# Autodesk Inventor assembly: sestava tělo estonsko s plechem otočené motory
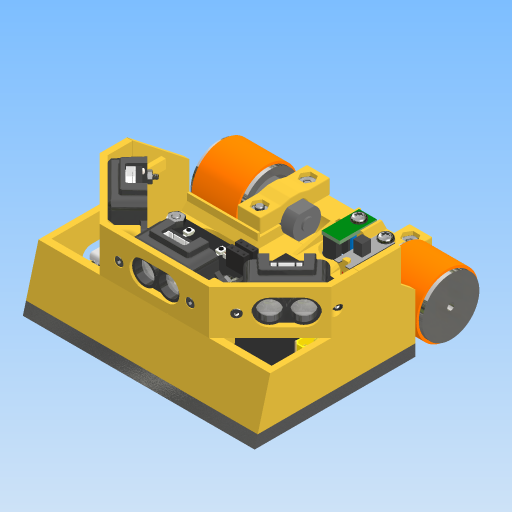
[picture p0: Inventor's stored thumbnail of the model, 512x512]
Saved by Autodesk Inventor 2024.2 (Build 282272000, 272)
## iProperties
Created: 2023-11-14
Part Number: sestava tělo estonsko s plechem otočené motory
Document SubType Name: Assembly
Designer: Simak
Author: Simak
## Documents named in this file (21)
- C:\Users\MenMe\Рабочий стол\GitHub\RoboCop\- 3D -\wip\Tělo s plechem\sestava tělo estonsko s plechem otočené motory.iam
- C:\Users\MenMe\Рабочий стол\GitHub\RoboCop\- 3D -\wip\Tělo s plechem\tělo estonsko s plechem otočené motory.ipt
- C:\Users\MenMe\Рабочий стол\GitHub\RoboCop\- 3D -\mech._parts\plech.ipt
- C:\Users\MenMe\Рабочий стол\GitHub\RoboCop\- 3D -\el._parts\sumec_smd.iam
- C:\Users\MenMe\Рабочий стол\GitHub\RoboCop\- 3D -\wip\Sestava TF-Luna a držáku.iam
- C:\Users\MenMe\Рабочий стол\GitHub\RoboCop\- 3D -\el._parts\qre_module.ipt
- C:\Users\MenMe\Рабочий стол\GitHub\RoboCop\- 3D -\el._parts\switch.ipt
- C:\Users\MenMe\Рабочий стол\GitHub\RoboCop\- 3D -\el._parts\GA12-N20_Motor.ipt
- C:\Users\MenMe\Рабочий стол\GitHub\RoboCop\- 3D -\mech._parts\wheel+silicon.ipt
- C:\Users\MenMe\Рабочий стол\GitHub\RoboCop\- 3D -\mech._parts\motor_C_clamp_nutt_motor_otoceny.ipt
- C:\Users\MenMe\Рабочий стол\GitHub\RoboCop\- 3D -\screws+nuts\Šrouby\M3_kuzel_torx\torx_socket_countersunk_flat_head_M3x18.ipt
- C:\Users\MenMe\Рабочий стол\GitHub\RoboCop\- 3D -\screws+nuts\matky\M3 Nut.ipt
- C:\Users\MenMe\Рабочий стол\GitHub\RoboCop\- 3D -\screws+nuts\Šrouby\M3_kuzel_torx\torx_socket_countersunk_flat_head_M3x08.ipt
- C:\Users\MenMe\Рабочий стол\GitHub\RoboCop\- 3D -\screws+nuts\Šrouby\M3_koule_torx\torx_socket_button_head_M3x08.ipt
- C:\Users\MenMe\Рабочий стол\GitHub\RoboCop\- 3D -\screws+nuts\Šrouby\M3_kuzel_torx\torx_socket_countersunk_flat_head_M3x12.ipt
- C:\Users\MenMe\Рабочий стол\GitHub\RoboCop\- 3D -\screws+nuts\Šrouby\M3_koule_torx\torx_socket_button_head_M3x10.ipt
- C:\Users\MenMe\Рабочий стол\GitHub\RoboCop\- 3D -\screws+nuts\Šrouby\M2_valec_imbus\M2 x 0.4mm Thread 16mm LONG SOCKET HEAD CAP SCREW.ipt
- C:\Users\MenMe\Рабочий стол\GitHub\RoboCop\- 3D -\screws+nuts\Šrouby\M2_valec_imbus\M2 x 0.4mm Thread 12mm LONG SOCKET HEAD CAP SCREW.ipt
- C:\Users\MenMe\Рабочий стол\GitHub\RoboCop\- 3D -\el._parts\connectors\XT30\XT30_Stecker.ipt
- C:\Users\MenMe\Рабочий стол\GitHub\RoboCop\- 3D -\screws+nuts\matky\M2 x 0.4mm Thread HEX NUT.ipt
- C:\Users\MenMe\Рабочий стол\GitHub\RoboCop\- 3D -\mech._parts\oddělovací plocha.ipt
## Components (50 placed, 20 different names)
1. tělo estonsko s plechem otočené motory:1 — Mate:1, Flush:1, Flush:2, Mate:2, Insert:1, Insert:2, Mate:3, Mate:4, Flush:3, Insert:3, Mate:5, Mate:6, Mate:7, Mate:8, Mate:10, Mate:11, Mate:12, Mate:13, Mate:14, Mate:15, Flush:4, Flush:5, Mate:19, Insert:4, Mate:21, Insert:5, Insert:8, Insert:9, Mate:28, Mate:39, Mate:40, Insert:27, Insert:28, Mate:41, Mate:42, Insert:34, Mate:45, Mate:47
2. plech:1 — Mate:1, Flush:1, Flush:2, Insert:6, Insert:7, Insert:11, Insert:12, Insert:13, Insert:14, Mate:46, Insert:35
3. sumec_smd:1 [sub-assembly] — Mate:2, Insert:1, Insert:2, Mate:34, Mate:35, Mate:36, Insert:23, Insert:24, Insert:25, Insert:26
4. Sestava TF-Luna a držáku:1 [sub-assembly] — Mate:3, Mate:4, Flush:3, Mate:30, Mate:31, Mate:32, Mate:33, Insert:15, Insert:16, Insert:17, Insert:18, Insert:19, Insert:20, Mate:44, Insert:29, Insert:30, Insert:31, Insert:32, Insert:33
5. qre_module:1 — Insert:3, Mate:5, Insert:10
6. switch:1 — Mate:6, Mate:7, Mate:8, Mate:29
7. GA12-N20_Motor:1 — Mate:13, Mate:14, Mate:15, Mate:17, Mate:20
8. GA12-N20_Motor:2 — Mate:10, Mate:11, Mate:12, Mate:16, Mate:18
9. wheel+silicon:1 — Flush:5, Mate:17
10. wheel+silicon:2 — Flush:4, Mate:16
11. motor_C_clamp_nutt_motor_otoceny:1 — Mate:18, Mate:19, Insert:4, Mate:22, Mate:24, Insert:21, Mate:37
12. motor_C_clamp_nutt_motor_otoceny:2 — Mate:20, Mate:21, Insert:5, Mate:25, Mate:27, Insert:22, Mate:38
13. torx_socket_countersunk_flat_head_M3x18:1 — Insert:7, Mate:23
14. torx_socket_countersunk_flat_head_M3x18:2 — Insert:6, Mate:26
15. M3 Nut:6 — Mate:25, Mate:26, Mate:27
16. M3 Nut:8 — Mate:22, Mate:23, Mate:24
17. torx_socket_countersunk_flat_head_M3x08:1 — Insert:9
18. torx_socket_countersunk_flat_head_M3x08:2 — Insert:8
19. torx_socket_button_head_M3x08:1 — Insert:10
20. torx_socket_button_head_M3x08:2 — Mate:28, Mate:29
21. torx_socket_countersunk_flat_head_M3x12:1 — Insert:14
22. torx_socket_countersunk_flat_head_M3x12:2 — Insert:12
23. torx_socket_countersunk_flat_head_M3x12:3 — Insert:13
24. torx_socket_countersunk_flat_head_M3x12:4 — Insert:11
25. torx_socket_button_head_M3x10:1 — Mate:31, Mate:32
26. torx_socket_button_head_M3x10:2 — Mate:30, Mate:33
27. M2 x 0.4mm Thread 16mm LONG SOCKET HEAD CAP SCREW:1 — Insert:18
28. M2 x 0.4mm Thread 16mm LONG SOCKET HEAD CAP SCREW:2 — Insert:17
29. M2 x 0.4mm Thread 16mm LONG SOCKET HEAD CAP SCREW:3 — Insert:16
30. M2 x 0.4mm Thread 16mm LONG SOCKET HEAD CAP SCREW:4 — Insert:15
31. M2 x 0.4mm Thread 12mm LONG SOCKET HEAD CAP SCREW:1 — Insert:20
32. M2 x 0.4mm Thread 12mm LONG SOCKET HEAD CAP SCREW:2 — Insert:19, Mate:43
33. XT30_Stecker:1 — Mate:34, Mate:35, Mate:36
34. M3 Nut:9 — Insert:24
35. M3 Nut:10 — Insert:23
36. M3 Nut:11 — Mate:39, Mate:40
37. M3 Nut:12 — Insert:21, Mate:37
38. M3 Nut:13 — Insert:22, Mate:38
39. M3 Nut:14 — Insert:25
40. M3 Nut:15 — Insert:26
41. M3 Nut:16 — Insert:28, Mate:41
42. M3 Nut:17 — Insert:27, Mate:42
43. M2 x 0.4mm Thread HEX NUT:1 — Insert:31
44. M2 x 0.4mm Thread HEX NUT:2 — Insert:30
45. M2 x 0.4mm Thread HEX NUT:3 — Insert:33
46. M2 x 0.4mm Thread HEX NUT:4 — Insert:32
47. M2 x 0.4mm Thread HEX NUT:5 — Insert:29
48. M2 x 0.4mm Thread HEX NUT:6 — Mate:43, Mate:44
49. M3 Nut:18 — Insert:34, Mate:45
50. oddělovací plocha:1 — Mate:46, Insert:35, Mate:47
## Relationships (86: Mate 46, Insert 35, Flush 5)
- Mate:1: tělo estonsko s plechem otočené motory:1 ↔ plech:1
- Flush:1: tělo estonsko s plechem otočené motory:1 ↔ plech:1
- Flush:2: tělo estonsko s plechem otočené motory:1 ↔ plech:1
- Mate:2: tělo estonsko s plechem otočené motory:1 ↔ sumec_smd:1
- Insert:1: tělo estonsko s plechem otočené motory:1 ↔ sumec_smd:1
- Insert:2: tělo estonsko s plechem otočené motory:1 ↔ sumec_smd:1
- Mate:3: tělo estonsko s plechem otočené motory:1 ↔ Sestava TF-Luna a držáku:1
- Mate:4: tělo estonsko s plechem otočené motory:1 ↔ Sestava TF-Luna a držáku:1
- Flush:3: tělo estonsko s plechem otočené motory:1 ↔ Sestava TF-Luna a držáku:1
- Insert:3: tělo estonsko s plechem otočené motory:1 ↔ qre_module:1
- Mate:5: tělo estonsko s plechem otočené motory:1 ↔ qre_module:1
- Mate:6: tělo estonsko s plechem otočené motory:1 ↔ switch:1
- Mate:7: tělo estonsko s plechem otočené motory:1 ↔ switch:1
- Mate:8: tělo estonsko s plechem otočené motory:1 ↔ switch:1
- Mate:10: tělo estonsko s plechem otočené motory:1 ↔ GA12-N20_Motor:2
- Mate:11: tělo estonsko s plechem otočené motory:1 ↔ GA12-N20_Motor:2
- Mate:12: tělo estonsko s plechem otočené motory:1 ↔ GA12-N20_Motor:2
- Mate:13: tělo estonsko s plechem otočené motory:1 ↔ GA12-N20_Motor:1
- Mate:14: tělo estonsko s plechem otočené motory:1 ↔ GA12-N20_Motor:1
- Mate:15: tělo estonsko s plechem otočené motory:1 ↔ GA12-N20_Motor:1
- Flush:4: tělo estonsko s plechem otočené motory:1 ↔ wheel+silicon:2
- Mate:16: GA12-N20_Motor:2 ↔ wheel+silicon:2
- Flush:5: tělo estonsko s plechem otočené motory:1 ↔ wheel+silicon:1
- Mate:17: GA12-N20_Motor:1 ↔ wheel+silicon:1
- Mate:18: GA12-N20_Motor:2 ↔ motor_C_clamp_nutt_motor_otoceny:1
- Mate:19: tělo estonsko s plechem otočené motory:1 ↔ motor_C_clamp_nutt_motor_otoceny:1
- Insert:4: tělo estonsko s plechem otočené motory:1 ↔ motor_C_clamp_nutt_motor_otoceny:1
- Mate:20: GA12-N20_Motor:1 ↔ motor_C_clamp_nutt_motor_otoceny:2
- Mate:21: tělo estonsko s plechem otočené motory:1 ↔ motor_C_clamp_nutt_motor_otoceny:2
- Insert:5: tělo estonsko s plechem otočené motory:1 ↔ motor_C_clamp_nutt_motor_otoceny:2
- Insert:6: plech:1 ↔ torx_socket_countersunk_flat_head_M3x18:2
- Insert:7: plech:1 ↔ torx_socket_countersunk_flat_head_M3x18:1
- Mate:22: motor_C_clamp_nutt_motor_otoceny:1 ↔ M3 Nut:8
- Mate:23: torx_socket_countersunk_flat_head_M3x18:1 ↔ M3 Nut:8
- Mate:24: motor_C_clamp_nutt_motor_otoceny:1 ↔ M3 Nut:8
- Mate:25: motor_C_clamp_nutt_motor_otoceny:2 ↔ M3 Nut:6
- Mate:26: torx_socket_countersunk_flat_head_M3x18:2 ↔ M3 Nut:6
- Mate:27: motor_C_clamp_nutt_motor_otoceny:2 ↔ M3 Nut:6
- Insert:8: tělo estonsko s plechem otočené motory:1 ↔ torx_socket_countersunk_flat_head_M3x08:2
- Insert:9: tělo estonsko s plechem otočené motory:1 ↔ torx_socket_countersunk_flat_head_M3x08:1
- Insert:10: qre_module:1 ↔ torx_socket_button_head_M3x08:1
- Mate:28: tělo estonsko s plechem otočené motory:1 ↔ torx_socket_button_head_M3x08:2
- Mate:29: switch:1 ↔ torx_socket_button_head_M3x08:2
- Insert:11: plech:1 ↔ torx_socket_countersunk_flat_head_M3x12:4
- Insert:12: plech:1 ↔ torx_socket_countersunk_flat_head_M3x12:2
- Insert:13: plech:1 ↔ torx_socket_countersunk_flat_head_M3x12:3
- Insert:14: plech:1 ↔ torx_socket_countersunk_flat_head_M3x12:1
- Mate:30: Sestava TF-Luna a držáku:1 ↔ torx_socket_button_head_M3x10:2
- Mate:31: Sestava TF-Luna a držáku:1 ↔ torx_socket_button_head_M3x10:1
- Mate:32: Sestava TF-Luna a držáku:1 ↔ torx_socket_button_head_M3x10:1
- Mate:33: Sestava TF-Luna a držáku:1 ↔ torx_socket_button_head_M3x10:2
- Insert:15: Sestava TF-Luna a držáku:1 ↔ M2 x 0.4mm Thread 16mm LONG SOCKET HEAD CAP SCREW:4
- Insert:16: Sestava TF-Luna a držáku:1 ↔ M2 x 0.4mm Thread 16mm LONG SOCKET HEAD CAP SCREW:3
- Insert:17: Sestava TF-Luna a držáku:1 ↔ M2 x 0.4mm Thread 16mm LONG SOCKET HEAD CAP SCREW:2
- Insert:18: Sestava TF-Luna a držáku:1 ↔ M2 x 0.4mm Thread 16mm LONG SOCKET HEAD CAP SCREW:1
- Insert:19: Sestava TF-Luna a držáku:1 ↔ M2 x 0.4mm Thread 12mm LONG SOCKET HEAD CAP SCREW:2
- Insert:20: Sestava TF-Luna a držáku:1 ↔ M2 x 0.4mm Thread 12mm LONG SOCKET HEAD CAP SCREW:1
- Mate:34: sumec_smd:1 ↔ XT30_Stecker:1
- Mate:35: sumec_smd:1 ↔ XT30_Stecker:1
- Mate:36: sumec_smd:1 ↔ XT30_Stecker:1
- Insert:21: motor_C_clamp_nutt_motor_otoceny:1 ↔ M3 Nut:12
- Mate:37: motor_C_clamp_nutt_motor_otoceny:1 ↔ M3 Nut:12
- Insert:22: motor_C_clamp_nutt_motor_otoceny:2 ↔ M3 Nut:13
- Mate:38: motor_C_clamp_nutt_motor_otoceny:2 ↔ M3 Nut:13
- Mate:39: tělo estonsko s plechem otočené motory:1 ↔ M3 Nut:11
- Mate:40: tělo estonsko s plechem otočené motory:1 ↔ M3 Nut:11
- Insert:23: sumec_smd:1 ↔ M3 Nut:10
- Insert:24: sumec_smd:1 ↔ M3 Nut:9
- Insert:25: sumec_smd:1 ↔ M3 Nut:14
- Insert:26: sumec_smd:1 ↔ M3 Nut:15
- Insert:27: tělo estonsko s plechem otočené motory:1 ↔ M3 Nut:17
- Insert:28: tělo estonsko s plechem otočené motory:1 ↔ M3 Nut:16
- Mate:41: tělo estonsko s plechem otočené motory:1 ↔ M3 Nut:16
- Mate:42: tělo estonsko s plechem otočené motory:1 ↔ M3 Nut:17
- Mate:43: M2 x 0.4mm Thread 12mm LONG SOCKET HEAD CAP SCREW:2 ↔ M2 x 0.4mm Thread HEX NUT:6
- Mate:44: Sestava TF-Luna a držáku:1 ↔ M2 x 0.4mm Thread HEX NUT:6
- Insert:29: Sestava TF-Luna a držáku:1 ↔ M2 x 0.4mm Thread HEX NUT:5
- Insert:30: Sestava TF-Luna a držáku:1 ↔ M2 x 0.4mm Thread HEX NUT:2
- Insert:31: Sestava TF-Luna a držáku:1 ↔ M2 x 0.4mm Thread HEX NUT:1
- Insert:32: Sestava TF-Luna a držáku:1 ↔ M2 x 0.4mm Thread HEX NUT:4
- Insert:33: Sestava TF-Luna a držáku:1 ↔ M2 x 0.4mm Thread HEX NUT:3
- Insert:34: tělo estonsko s plechem otočené motory:1 ↔ M3 Nut:18
- Mate:45: tělo estonsko s plechem otočené motory:1 ↔ M3 Nut:18
- Mate:46: plech:1 ↔ oddělovací plocha:1
- Insert:35: plech:1 ↔ oddělovací plocha:1
- Mate:47: tělo estonsko s plechem otočené motory:1 ↔ oddělovací plocha:1
